# Autodesk Inventor assembly: PowerSupply
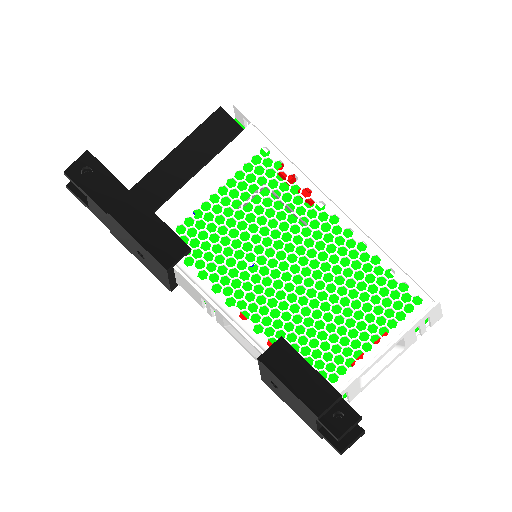
[picture p0: Inventor's stored thumbnail of the model, 512x512]
Saved by Autodesk Inventor 2025.2 (Build 292293000, 293)
## iProperties
Created: 2026-03-31
Part Number: PowerSupply
Document SubType Name: Assembly
Designer: rolan
Author: rolan
## Documents named in this file (4)
- C:\Users\rolan\Documents\PhD\Inventor\Assembly\PowerSupply.iam
- C:\Users\rolan\Documents\PhD\Inventor\Assembly\180992207-9-rsp-100-5\rsp-100-5.iam
- C:\Users\rolan\Documents\PhD\Inventor\Parts\PowerSupplyAttach.ipt
- C:\Users\rolan\Documents\PhD\Inventor\Parts\PowerSupplyAttachTop.ipt
## Components (3 placed, 3 different names)
1. rsp-100-5:1 [sub-assembly] — Mate:1, Mate:2, Mate:3, Mate:4, Mate:5, Mate:6
2. PowerSupplyAttach:1 — Mate:4, Mate:5, Mate:6
3. PowerSupplyAttachTop:1 — Mate:1, Mate:2, Mate:3
## Relationships (6: Mate 6)
- Mate:1: rsp-100-5:1 ↔ PowerSupplyAttachTop:1
- Mate:2: rsp-100-5:1 ↔ PowerSupplyAttachTop:1
- Mate:3: rsp-100-5:1 ↔ PowerSupplyAttachTop:1
- Mate:4: rsp-100-5:1 ↔ PowerSupplyAttach:1
- Mate:5: rsp-100-5:1 ↔ PowerSupplyAttach:1
- Mate:6: rsp-100-5:1 ↔ PowerSupplyAttach:1
